# Autodesk Inventor assembly: OpenFrame
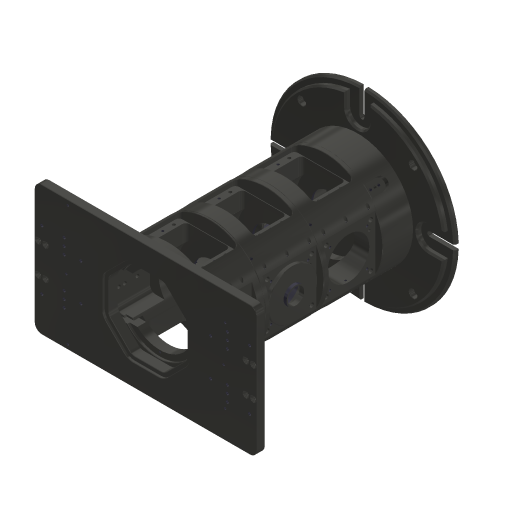
[picture p0: Inventor's stored thumbnail of the model, 512x512]
Saved by Autodesk Inventor 2024.1 (Build 281209000, 209)
## iProperties
Created: 2024-05-19
Part Number: OpenFrame
Document SubType Name: Assembly
Designer: AdminForWorker
Title: OpenFrame v1
Author: AdminForWorker
## Documents named in this file (7)
- C:\Users\diederichbenedict\Dropbox\Dokumente\Promotion\PROJECTS\SIMMO\INVENTOR\OpenFrame v1\OpenFrame.iam
- C:\Users\diederichbenedict\Dropbox\Dokumente\Promotion\PROJECTS\SIMMO\INVENTOR\OpenFrame v1\OF-LL-BP v1.ipt
- C:\Users\diederichbenedict\Dropbox\Dokumente\Promotion\PROJECTS\SIMMO\INVENTOR\OpenFrame v1\OpenFrame v1.iam
- C:\Users\diederichbenedict\Dropbox\Dokumente\Promotion\PROJECTS\SIMMO\INVENTOR\OpenFrame v1\OF-LL-FL-MOT v1.ipt
- C:\Users\diederichbenedict\Dropbox\Dokumente\Promotion\PROJECTS\SIMMO\INVENTOR\OpenFrame v1\OF-AD-SBSM2-CM v1.ipt
- C:\Users\diederichbenedict\Dropbox\Dokumente\Promotion\PROJECTS\SIMMO\INVENTOR\OpenFrame v1\OF-IN-MCH v1.ipt
- C:\Users\diederichbenedict\Dropbox\Dokumente\Promotion\PROJECTS\SIMMO\INVENTOR\OpenFrame v1\OF-LL-SP v1.ipt
## Components (8 placed, 6 different names)
1. OpenFrame v1:1 [sub-assembly] — Einfügen:1
2. OF-LL-FL-MOT v1:1
3. OF-AD-SBSM2-CM v1:1
4. OF-IN-MCH v1:1
5. OF-LL-SP v1:1
6. OF-LL-BP v1:1 — Einfügen:2
7. OpenFrame v1:2 [sub-assembly] — Einfügen:1, Einfügen:2, Einfügen:3
8. OF-AD-SBSM2-CM v1:2 — Einfügen:3
## Relationships (3: Insert 3)
- Einfügen:1 [Insert]: OpenFrame v1:1 ↔ OpenFrame v1:2
- Einfügen:2 [Insert]: OF-LL-BP v1:1 ↔ OpenFrame v1:2
- Einfügen:3 [Insert]: OpenFrame v1:2 ↔ OF-AD-SBSM2-CM v1:2
